# Autodesk Inventor assembly: Custom Vice V1
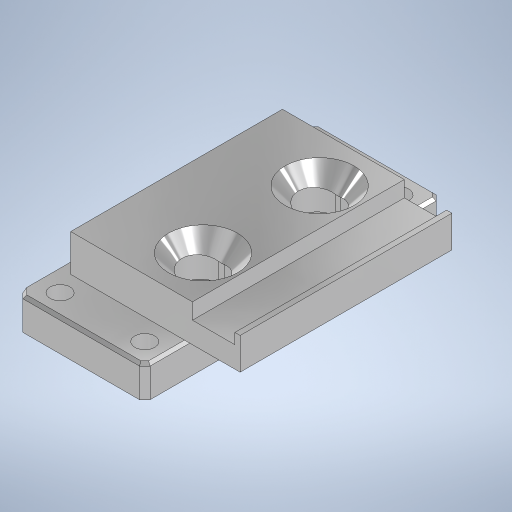
[picture p0: Inventor's stored thumbnail of the model, 512x512]
Saved by Autodesk Inventor 2023.2 (Build 272271000, 271)
## iProperties
Created: 2024-03-01
Part Number: Custom Vice V1
Document SubType Name: Assembly
Designer: Nathan Cai
Author: Nathan Cai
## Documents named in this file (3)
- E:\Documents\Inventor\Custom Vice V1\Custom Vice V1.iam
- E:\Documents\Inventor\Custom Vice V1\Base - Stationary.ipt
- E:\Documents\Inventor\Custom Vice V1\Jaw.ipt
## Components (2 placed, 2 different names)
1. Base - Stationary:1 — Mate:1, Mate:2, Mate:3
2. Jaw:1 — Mate:1, Mate:2, Mate:3
## Relationships (3: Mate 3)
- Mate:1: Base - Stationary:1 ↔ Jaw:1
- Mate:2: Base - Stationary:1 ↔ Jaw:1
- Mate:3: Base - Stationary:1 ↔ Jaw:1
